# Autodesk Inventor assembly: GP6-200
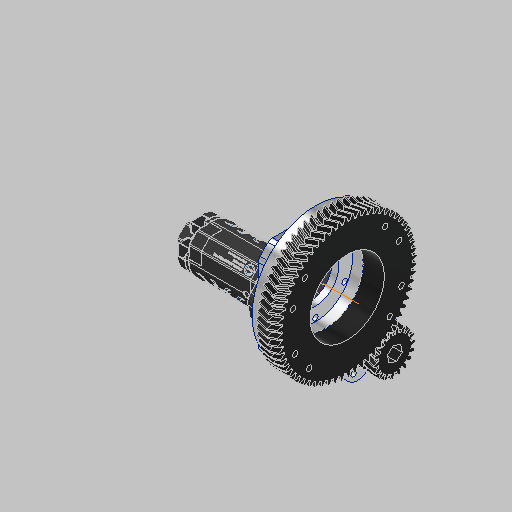
[picture p0: Inventor's stored thumbnail of the model, 512x512]
Saved by Autodesk Inventor 2023.5 (Build 275446000, 446)
## iProperties
Created: 2025-02-23
Part Number: GP6-200
Document SubType Name: Assembly
Designer: brand
Author: brand
## Documents named in this file (6)
- C:\Users\slick\OneDrive\Desktop\2025-ReefScape---CAD\Gripper\GP6\GP6-200.iam
- C:\Users\slick\OneDrive\Desktop\2025-ReefScape---CAD\Gripper\GP6\GP6-004.ipt
- C:\Users\slick\OneDrive\Desktop\2025-ReefScape---CAD\COMMON PARTS\4in Lazy Suzan.iam
- C:\Users\slick\OneDrive\Desktop\2025-ReefScape---CAD\COMMON PARTS\GEARS\Herringbone\2m 64t herringbone\2m 64t herringbone.ipt
- C:\Users\slick\OneDrive\Desktop\2025-ReefScape---CAD\COMMON PARTS\GEARBOXES\MAX Planetary\MAX Planetary Configurable 9-1 Kraken x44\MAX Planetary Configurable 9-1 Kraken x44.iam
- C:\Users\slick\OneDrive\Desktop\2025-ReefScape---CAD\COMMON PARTS\GEARS\Herringbone\2m 18t herringbone\2m 18t herringbone.ipt
## Components (5 placed, 5 different names)
1. GP6-004:1 — Mate:1
2. 4in Lazy Suzan:1 [sub-assembly] — Rotation:1
3. 2m 64t herringbone:1 — Flush:1
4. MAX Planetary Configurable 9-1 Kraken x44:1 [sub-assembly]
5. 2m 18t herringbone:1 — Mate:1, Flush:1, Rotation:1
## Relationships (9: Insert 6, Mate 1, Flush 1, RelateRotation 1)
- [Insert]: GP6-004:1 ↔ 4in Lazy Suzan:1
- [Insert]: GP6-004:1 ↔ 4in Lazy Suzan:1
- [Insert]: 4in Lazy Suzan:1 ↔ 2m 64t herringbone:1
- [Insert]: 4in Lazy Suzan:1 ↔ 2m 64t herringbone:1
- Mate:1: GP6-004:1 ↔ 2m 18t herringbone:1
- [Insert]: GP6-004:1 ↔ MAX Planetary Configurable 9-1 Kraken x44:1
- [Insert]: GP6-004:1 ↔ MAX Planetary Configurable 9-1 Kraken x44:1
- Flush:1: 2m 64t herringbone:1 ↔ 2m 18t herringbone:1
- Rotation:1 [RelateRotation] (3.5556 ul): 4in Lazy Suzan:1 ↔ 2m 18t herringbone:1
